# Autodesk Inventor assembly: PLA_Konrad_Kosugesnapshot7
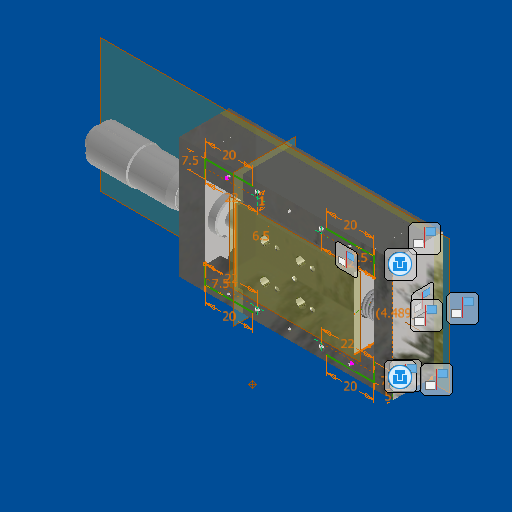
[picture p0: Inventor's stored thumbnail of the model, 512x512]
Saved by Autodesk Inventor 2025.1 (Build 291241000, 241)
## iProperties
Company: Politechnika Warszawska
Created: 2024-12-11
Part Number: PLA_Konrad_Kosugesnapshot7
Document SubType Name: Assembly
Designer: Konrad Kosuge
Engineer: Konrad Kosuge
Author: Konrad Kosuge
Title: Linear Stage Unit
## Documents named in this file (13)
- C:\Users\konch\OneDrive\Desktop\FMD_Konrad_Kosuge\PLA_Konrad_Kosugesnapshot7.iam
- C:\Users\konch\OneDrive\Desktop\FMD_Konrad_Kosuge\Micrometer_Head.ipt
- C:\Users\konch\OneDrive\Desktop\FMD_Konrad_Kosuge\Ball_Spacers.ipt
- C:\Users\konch\OneDrive\Desktop\FMD_Konrad_Kosuge\Guides.ipt
- C:\Users\konch\OneDrive\Desktop\FMD_Konrad_Kosuge\case.ipt
- C:\Users\konch\OneDrive\Desktop\FMD_Konrad_Kosuge\ending.ipt
- C:\Users\konch\OneDrive\Desktop\FMD_Konrad_Kosuge\Micrometer_Holder.ipt
- C:\Users\konch\OneDrive\Desktop\FMD_Konrad_Kosuge\platform_v2_slot.ipt
- C:\Users\konch\OneDrive\Desktop\FMD_Konrad_Kosuge\4mmBearing_CPY.ipt
- C:\Users\konch\OneDrive\Desktop\FMD_Konrad_Kosuge\Sodemann11980.ipt
- C:\Users\konch\OneDrive\Documents\Inventor\Content Center Files\R2025\en-US\ISO 4762(2)\ISO 4762 - M2 x 8ISO.ipt
- C:\Users\konch\OneDrive\Documents\Inventor\Content Center Files\R2025\en-US\ISO 4762(2)\ISO 4762 - M2 x 16ISO.ipt
- C:\Users\konch\OneDrive\Desktop\FMD_Konrad_Kosuge\ISO 2338 - 2 h8 x 10.ipt
## Components (36 placed, 12 different names)
1. Ball_Spacers:1 — Mate:26, Mate:27, Mate:49, Mate:50, Flush:2, Mate:54
2. Guides:2 — Mate:41, Mate:42, Mate:51, Mate:52, Mate:53
3. Guides:3 — Mate:39, Mate:47, Mate:49, Mate:50, Flush:1
4. case:1 — Mate:6, Mate:7, Mate:39, Mate:41, Mate:46, Mate:48, Rotational:1, Rotational:2, Rotational:3, Rotational:6, Insert:13, Rotational:7, Rotational:8, Rotational:9, Rotational:10, Rotational:11
5. ending:1 — Mate:7, Mate:36, Mate:42, Mate:43, Mate:44, Mate:47, Mate:48, Insert:9, Insert:10
6. Micrometer_Head:1 — Insert:1
7. Micrometer_Holder:1 — Insert:1, Mate:6, Mate:46, Insert:11, Insert:12
8. platform_v2_slot:1 — Mate:26, Mate:27, Mate:34, Tangent:13, Tangent:14, Mate:35, Mate:51, Flush:1, Flush:3
9. Ball_Spacers:2 — Mate:33, Mate:34, Mate:35, Mate:52, Mate:53, Flush:2, Flush:3
10. Sodemann11980:1 — Mate:36, Mate:43
11. ISO 4762 M2 x 8:7 — Insert:9
12. ISO 4762 M2 x 8:8 — Insert:10
13. ISO 4762 M2 x 16:3 — Insert:11
14. ISO 4762 M2 x 16:4 — Insert:12
15. ISO 4762 M2 x 8:10 — Rotational:2
16. ISO 4762 M2 x 8:11 — Rotational:3
17. ISO 4762 M2 x 8:12 — Rotational:6
18. ISO 4762 M2 x 8:13 — Rotational:1
19. ISO 2338 2 h8 x 10:1 — Insert:13
20. ISO 2338 2 h8 x 10:2 — Rotational:7
21. ISO 2338 2 h8 x 10:8 — Rotational:9
22. ISO 2338 2 h8 x 10:10 — Rotational:8
23. ISO 4762 M2 x 8:14 — Rotational:10
24. ISO 4762 M2 x 8:15 — Rotational:11
25. 4mmBearing_CPY:5 — Mate:33, Tangent:13, Tangent:14, Mate:54
26. 4mmBearing_CPY:6
27. 4mmBearing_CPY:7
28. 4mmBearing_CPY:8
29. 4mmBearing_CPY:9
30. 4mmBearing_CPY:10
31. 4mmBearing_CPY:11
32. 4mmBearing_CPY:12
33. 4mmBearing_CPY:13
34. 4mmBearing_CPY:14
35. 4mmBearing_CPY:15
36. 4mmBearing_CPY:16
## Component patterns: (12 elements, first: 4mmBearing_CPY:5)
## Relationships (42: Mate 22, RevoluteJoint 9, Insert 6, Flush 3, Tangent 2)
- Insert:1: Micrometer_Head:1 ↔ Micrometer_Holder:1
- Mate:6: case:1 ↔ Micrometer_Holder:1
- Mate:7: case:1 ↔ ending:1
- Mate:26: Ball_Spacers:1 ↔ platform_v2_slot:1
- Mate:27 (0.5 mm): Ball_Spacers:1 ↔ platform_v2_slot:1
- Mate:33: Ball_Spacers:2 ↔ 4mmBearing_CPY:5
- Mate:34: platform_v2_slot:1 ↔ Ball_Spacers:2
- Tangent:13: platform_v2_slot:1 ↔ 4mmBearing_CPY:5
- Tangent:14: platform_v2_slot:1 ↔ 4mmBearing_CPY:5
- Mate:35 (0.5 mm): platform_v2_slot:1 ↔ Ball_Spacers:2
- Mate:36: ending:1 ↔ Sodemann11980:1
- Mate:39: Guides:3 ↔ case:1
- Mate:41: Guides:2 ↔ case:1
- Mate:42: Guides:2 ↔ ending:1
- Mate:43: ending:1 ↔ Sodemann11980:1
- Mate:44: ending:1
- Mate:46: case:1 ↔ Micrometer_Holder:1
- Mate:47: Guides:3 ↔ ending:1
- Mate:48: case:1 ↔ ending:1
- Mate:49: Ball_Spacers:1 ↔ Guides:3
- Mate:50 (0.75 mm): Ball_Spacers:1 ↔ Guides:3
- Mate:51 (0.5 mm): Guides:2 ↔ platform_v2_slot:1
- Flush:1 (-2 mm): Guides:3 ↔ platform_v2_slot:1
- Mate:52: Guides:2 ↔ Ball_Spacers:2
- Mate:53 (0.75 mm): Guides:2 ↔ Ball_Spacers:2
- Flush:2: Ball_Spacers:1 ↔ Ball_Spacers:2
- Mate:54: Ball_Spacers:1 ↔ 4mmBearing_CPY:5
- Flush:3: platform_v2_slot:1 ↔ Ball_Spacers:2
- Insert:9: ending:1 ↔ ISO 4762 M2 x 8:7
- Insert:10: ending:1 ↔ ISO 4762 M2 x 8:8
- Insert:11: Micrometer_Holder:1 ↔ ISO 4762 M2 x 16:3
- Insert:12: Micrometer_Holder:1 ↔ ISO 4762 M2 x 16:4
- Rotational:1 [RevoluteJoint]: case:1 ↔ ISO 4762 M2 x 8:13
- Rotational:2 [RevoluteJoint]: case:1 ↔ ISO 4762 M2 x 8:10
- Rotational:3 [RevoluteJoint]: case:1 ↔ ISO 4762 M2 x 8:11
- Rotational:6 [RevoluteJoint]: case:1 ↔ ISO 4762 M2 x 8:12
- Insert:13: case:1 ↔ ISO 2338 2 h8 x 10:1
- Rotational:7 [RevoluteJoint]: case:1 ↔ ISO 2338 2 h8 x 10:2
- Rotational:8 [RevoluteJoint]: case:1 ↔ ISO 2338 2 h8 x 10:10
- Rotational:9 [RevoluteJoint]: case:1 ↔ ISO 2338 2 h8 x 10:8
- Rotational:10 [RevoluteJoint]: case:1 ↔ ISO 4762 M2 x 8:14
- Rotational:11 [RevoluteJoint]: case:1 ↔ ISO 4762 M2 x 8:15
